# Autodesk Inventor assembly: Sessao8_07_04_2025_999_0001
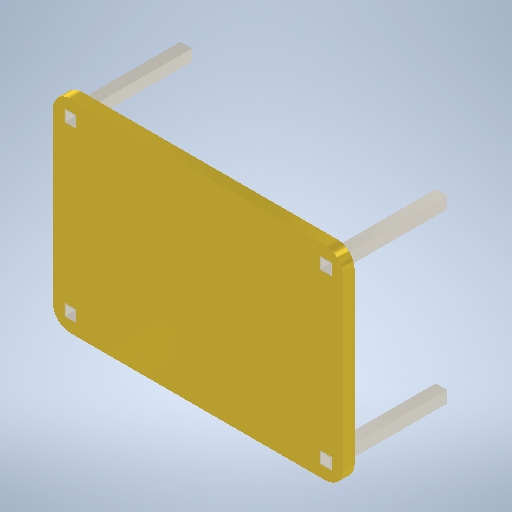
[picture p0: Inventor's stored thumbnail of the model, 512x512]
Saved by Autodesk Inventor 2025.2 (Build 292293000, 293)
## iProperties
Created: 2025-04-07
Part Number: Sessao8_07_04_2025_999_0001
Document SubType Name: Assembly
Designer: Gustavo Sousa
Author: Gustavo Sousa
## Documents named in this file (3)
- C:\Users\lucas\OneDrive\Documentos\Documentos\Gustavo\Mozangao\Robotica_Fundamentos\Inventor\Sessao8_07_04_2025\Sessao8_07_04_2025_999_0001.iam
- C:\Users\lucas\OneDrive\Documentos\Documentos\Gustavo\Mozangao\Robotica_Fundamentos\Inventor\Sessao8_07_04_2025\Sessao8_07_04_2025_0001_0001.ipt
- C:\Users\lucas\OneDrive\Documentos\Documentos\Gustavo\Mozangao\Robotica_Fundamentos\Inventor\Sessao8_07_04_2025\Sessao8_07_04_2025_0002_0001.ipt
## Components (5 placed, 2 different names)
1. Sessao8_07_04_2025_0001_0001:1 — Alinhado:1, Alinhado:2, Alinhado:3, Alinhado:4, Coincidente:2, Alinhado:10, Alinhado:11, Alinhado:12, Alinhado:13
2. Sessao8_07_04_2025_0002_0001:1 — Alinhado:6, Alinhado:8, Simetria:2, Alinhado:12
3. Sessao8_07_04_2025_0002_0001:2 — Alinhado:7, Alinhado:8, Alinhado:13
4. Sessao8_07_04_2025_0002_0001:3 — Alinhado:5, Alinhado:7, Alinhado:9, Simetria:1, Alinhado:11
5. Sessao8_07_04_2025_0002_0001:4 — Alinhado:4, Coincidente:2, Alinhado:5, Alinhado:6, Alinhado:9, Simetria:1, Simetria:2, Alinhado:10
## Relationships (16: Flush 13, Symmetry 2, Mate 1)
- Alinhado:1 [Flush]: Sessao8_07_04_2025_0001_0001:1
- Alinhado:2 [Flush]: Sessao8_07_04_2025_0001_0001:1
- Alinhado:3 [Flush]: Sessao8_07_04_2025_0001_0001:1
- Alinhado:4 [Flush] (30 mm): Sessao8_07_04_2025_0001_0001:1 ↔ Sessao8_07_04_2025_0002_0001:4
- Coincidente:2 [Mate] (-30 mm): Sessao8_07_04_2025_0001_0001:1 ↔ Sessao8_07_04_2025_0002_0001:4
- Alinhado:5 [Flush]: Sessao8_07_04_2025_0002_0001:3 ↔ Sessao8_07_04_2025_0002_0001:4
- Alinhado:6 [Flush]: Sessao8_07_04_2025_0002_0001:1 ↔ Sessao8_07_04_2025_0002_0001:4
- Alinhado:7 [Flush]: Sessao8_07_04_2025_0002_0001:2 ↔ Sessao8_07_04_2025_0002_0001:3
- Alinhado:8 [Flush]: Sessao8_07_04_2025_0002_0001:1 ↔ Sessao8_07_04_2025_0002_0001:2
- Alinhado:9 [Flush]: Sessao8_07_04_2025_0002_0001:3 ↔ Sessao8_07_04_2025_0002_0001:4
- Simetria:1 [Symmetry]: Sessao8_07_04_2025_0002_0001:3 ↔ Sessao8_07_04_2025_0002_0001:4
- Simetria:2 [Symmetry]: Sessao8_07_04_2025_0002_0001:1 ↔ Sessao8_07_04_2025_0002_0001:4
- Alinhado:10 [Flush]: Sessao8_07_04_2025_0001_0001:1 ↔ Sessao8_07_04_2025_0002_0001:4
- Alinhado:11 [Flush]: Sessao8_07_04_2025_0001_0001:1 ↔ Sessao8_07_04_2025_0002_0001:3
- Alinhado:12 [Flush]: Sessao8_07_04_2025_0001_0001:1 ↔ Sessao8_07_04_2025_0002_0001:1
- Alinhado:13 [Flush]: Sessao8_07_04_2025_0001_0001:1 ↔ Sessao8_07_04_2025_0002_0001:2
